# Autodesk Inventor assembly: HbMRLFinger
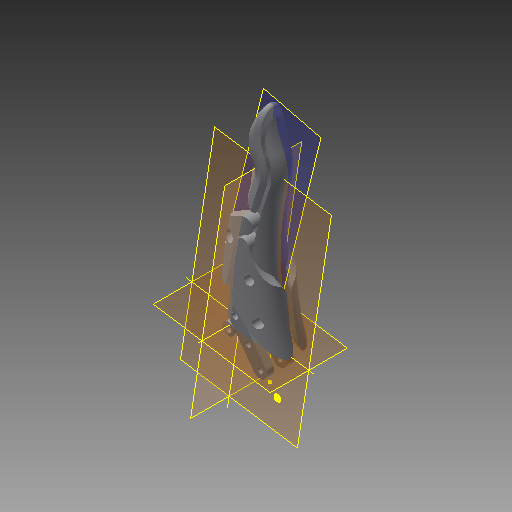
[picture p0: Inventor's stored thumbnail of the model, 512x512]
Saved by Autodesk Inventor 2018.1 (Build 221171000, 171)
## iProperties
Part Number: HbMRLFinger
Material: 一般
Document SubType Name: Assembly
Designer: sktom
Author: sktom
## Documents named in this file (7)
- D:\CloudStrage\OneDrive\CAD\MAJ\hackberry\HACKberry-hardware\3D_69%inlength\Inventor\HbHandForChild\HbFinger01ForChild\HbFinger01ForChild.iam
- D:\CloudStrage\OneDrive\CAD\MAJ\hackberry\HACKberry-hardware\3D_69%inlength\Inventor\HbHandForChild\HbFinger01ForChild\HbCouplerLinkCover03ForChild.ipt
- D:\CloudStrage\OneDrive\CAD\MAJ\hackberry\HACKberry-hardware\3D_69%inlength\Inventor\HbHandForChild\HbFinger01ForChild\HbCouplerLink02ForChild.ipt
- D:\CloudStrage\OneDrive\CAD\MAJ\hackberry\HACKberry-hardware\3D_69%inlength\Inventor\HbHandForChild\HbFinger01ForChild\HbMiddle-DistalPhalanx02ForChild.ipt
- D:\CloudStrage\OneDrive\CAD\MAJ\hackberry\HACKberry-hardware\3D_69%inlength\Inventor\HbHandForChild\HbFinger01ForChild\HbProximalPhalanx02ForChild.ipt
- D:\CloudStrage\OneDrive\CAD\MAJ\hackberry\HACKberry-hardware\3D_69%inlength\Inventor\HbHandForChild\HbFinger01ForChild\HbProximalPhalanxCover02ForChild.ipt
- D:\CloudStrage\OneDrive\CAD\MAJ\hackberry\HACKberry-hardware\3D_69%inlength\Inventor\HbHandForChild\HbFinger01ForChild\shaft_phi1.5_l6.ipt
## Components (7 placed, 6 different names)
1. HbCouplerLinkCover03ForChild:1 — 挿入:1, 挿入:2
2. HbCouplerLink02ForChild:1 — 挿入:1, 挿入:2, 挿入:3, 挿入:8
3. HbMiddle-DistalPhalanx02ForChild:1 — 挿入:3, 挿入:4, 円柱状:1, 円柱状:2
4. HbProximalPhalanx02ForChild:1 — 挿入:5, 挿入:6
5. HbProximalPhalanxCover02ForChild:1 — 挿入:4, 挿入:5, 挿入:6, 挿入:7
6. shaft_phi1.5_l6:1 — 円柱状:1, 挿入:7
7. shaft_phi1.5_l6:2 — 円柱状:2, 挿入:8
## Relationships (10: Insert 8, CylindricalJoint 2)
- 挿入:1 [Insert]: HbCouplerLinkCover03ForChild:1 ↔ HbCouplerLink02ForChild:1
- 挿入:2 [Insert]: HbCouplerLinkCover03ForChild:1 ↔ HbCouplerLink02ForChild:1
- 挿入:3 [Insert] (0.4 mm): HbCouplerLink02ForChild:1 ↔ HbMiddle-DistalPhalanx02ForChild:1
- 挿入:4 [Insert] (0.4 mm): HbMiddle-DistalPhalanx02ForChild:1 ↔ HbProximalPhalanxCover02ForChild:1
- 挿入:5 [Insert]: HbProximalPhalanx02ForChild:1 ↔ HbProximalPhalanxCover02ForChild:1
- 挿入:6 [Insert]: HbProximalPhalanx02ForChild:1 ↔ HbProximalPhalanxCover02ForChild:1
- 円柱状:1 [CylindricalJoint]: HbMiddle-DistalPhalanx02ForChild:1 ↔ shaft_phi1.5_l6:1
- 円柱状:2 [CylindricalJoint]: HbMiddle-DistalPhalanx02ForChild:1 ↔ shaft_phi1.5_l6:2
- 挿入:7 [Insert] (0.5 mm): HbProximalPhalanxCover02ForChild:1 ↔ shaft_phi1.5_l6:1
- 挿入:8 [Insert] (0.5 mm): HbCouplerLink02ForChild:1 ↔ shaft_phi1.5_l6:2
